# Autodesk Inventor assembly: richHolder
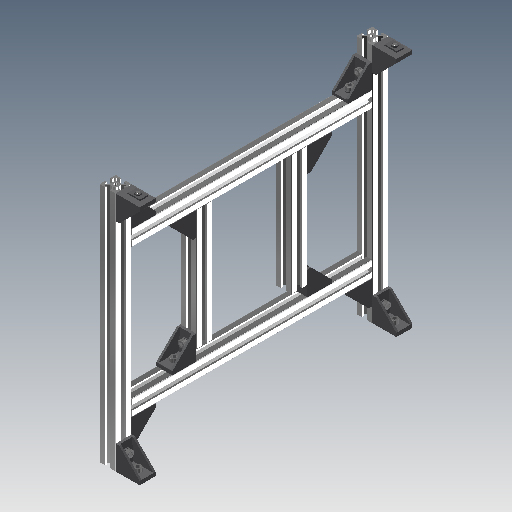
[picture p0: Inventor's stored thumbnail of the model, 512x512]
Saved by Autodesk Inventor 2018.2 (Build 222227000, 227)
## iProperties
Created: 2016-02-08
Part Number: richHolder
Document SubType Name: Assembly
Designer: Sawaiz
Author: Sawaiz
## Documents named in this file (6)
- C:\Users\sawaiz\OneDrive\projects\modularRICHFrame\frame\richHolder.iam
- C:\Users\sawaiz\OneDrive\projects\modularRICHFrame\hardware\angleBracket.iam
- C:\Users\sawaiz\OneDrive\projects\modularRICHFrame\frame\hfs5-2020Height.ipt
- C:\Users\sawaiz\OneDrive\projects\modularRICHFrame\frame\hfs5-2020Width.ipt
- C:\Users\sawaiz\OneDrive\projects\modularRICHFrame\frame\hfs5-2020BoxSeperator.ipt
- C:\Users\sawaiz\OneDrive\projects\modularRICHFrame\modularRICHFrame.xlsx
## Components (18 placed, 4 different names)
1. angleBracket:1 [sub-assembly] — Flush:30, Flush:31, Flush:35, Mate:19
2. angleBracket:2 [sub-assembly] — Flush:42, Flush:43, Mate:20
3. angleBracket:3 [sub-assembly] — Symmetry:4, Flush:33, Flush:34, Mate:21
4. angleBracket:4 [sub-assembly] — Symmetry:4, Flush:41, Flush:44, Mate:22
5. angleBracket:5 [sub-assembly] — Flush:6, Flush:7, Flush:10, Flush:12, Flush:32, Flush:50, Mate:24
6. angleBracket:6 [sub-assembly] — Flush:6, Flush:10, Flush:13, Flush:45, Flush:51, Mate:23
7. angleBracket:7 [sub-assembly] — Flush:5, Flush:7, Flush:9, Flush:12, Flush:36, Flush:48
8. angleBracket:8 [sub-assembly] — Flush:5, Flush:9, Flush:13, Flush:46, Flush:49, Mate:25
9. hfs5-2020Height:1 — Flush:30, Flush:31, Flush:42, Flush:43, Mate:19, Mate:20, Flush:47, Symmetry:5, Mate:26, Flush:52, Symmetry:8
10. hfs5-2020Height:2 — Flush:33, Flush:34, Flush:35, Flush:41, Flush:44, Mate:21, Mate:22, Flush:47, Symmetry:5, Mate:27, Symmetry:8
11. hfs5-2020Width:1 — Flush:45, Flush:46, Flush:49, Flush:51, Symmetry:6, Mate:23, Mate:25, Mate:31
12. hfs5-2020Width:2 — Flush:32, Flush:36, Flush:48, Flush:50, Symmetry:6, Mate:24, Mate:26, Mate:27, Flush:52, Flush:63, Mate:30
13. angleBracket:9 [sub-assembly] — Flush:22, Flush:26, Flush:39, Flush:54, Flush:55, Flush:61, Mate:29
14. angleBracket:10 [sub-assembly] — Flush:22, Flush:26, Flush:37, Flush:53, Flush:56, Flush:62, Mate:28
15. angleBracket:11 [sub-assembly] — Flush:24, Flush:27, Flush:40, Flush:54, Flush:60, Mate:31
16. angleBracket:12 [sub-assembly] — Flush:24, Flush:27, Flush:38, Flush:53, Flush:59
17. hfs5-2020BoxSeperator:1 — Flush:39, Flush:40, Symmetry:7, Flush:55, Flush:60, Flush:61, Mate:29
18. hfs5-2020BoxSeperator:2 — Flush:37, Flush:38, Symmetry:7, Flush:56, Flush:59, Flush:62, Mate:28, Flush:63, Mate:30
## Relationships (61: Flush 43, Mate 13, Symmetry 5)
- Flush:5: angleBracket:7 ↔ angleBracket:8
- Flush:6: angleBracket:5 ↔ angleBracket:6
- Flush:7: angleBracket:5 ↔ angleBracket:7
- Flush:9: angleBracket:7 ↔ angleBracket:8
- Flush:10: angleBracket:5 ↔ angleBracket:6
- Flush:12: angleBracket:5 ↔ angleBracket:7
- Flush:13: angleBracket:6 ↔ angleBracket:8
- Flush:22: angleBracket:9 ↔ angleBracket:10
- Flush:24: angleBracket:11 ↔ angleBracket:12
- Flush:26: angleBracket:9 ↔ angleBracket:10
- Flush:27: angleBracket:11 ↔ angleBracket:12
- Symmetry:4: angleBracket:3 ↔ angleBracket:4
- Flush:30: angleBracket:1 ↔ hfs5-2020Height:1
- Flush:31: angleBracket:1 ↔ hfs5-2020Height:1
- Flush:32: angleBracket:5 ↔ hfs5-2020Width:2
- Flush:33: angleBracket:3 ↔ hfs5-2020Height:2
- Flush:34: angleBracket:3 ↔ hfs5-2020Height:2
- Flush:35: angleBracket:1 ↔ hfs5-2020Height:2
- Flush:36: angleBracket:7 ↔ hfs5-2020Width:2
- Flush:37: angleBracket:10 ↔ hfs5-2020BoxSeperator:2
- Flush:38: angleBracket:12 ↔ hfs5-2020BoxSeperator:2
- Flush:39: angleBracket:9 ↔ hfs5-2020BoxSeperator:1
- Flush:40: angleBracket:11 ↔ hfs5-2020BoxSeperator:1
- Flush:41: angleBracket:4 ↔ hfs5-2020Height:2
- Flush:42: angleBracket:2 ↔ hfs5-2020Height:1
- Flush:43: angleBracket:2 ↔ hfs5-2020Height:1
- Flush:44: angleBracket:4 ↔ hfs5-2020Height:2
- Flush:45: angleBracket:6 ↔ hfs5-2020Width:1
- Flush:46: angleBracket:8 ↔ hfs5-2020Width:1
- Mate:19: angleBracket:1 ↔ hfs5-2020Height:1
- Mate:20: angleBracket:2 ↔ hfs5-2020Height:1
- Mate:21: angleBracket:3 ↔ hfs5-2020Height:2
- Mate:22: angleBracket:4 ↔ hfs5-2020Height:2
- Flush:47: hfs5-2020Height:1 ↔ hfs5-2020Height:2
- Symmetry:5: hfs5-2020Height:1 ↔ hfs5-2020Height:2
- Flush:48: angleBracket:7 ↔ hfs5-2020Width:2
- Flush:49: angleBracket:8 ↔ hfs5-2020Width:1
- Flush:50: angleBracket:5 ↔ hfs5-2020Width:2
- Flush:51: angleBracket:6 ↔ hfs5-2020Width:1
- Symmetry:6: hfs5-2020Width:1 ↔ hfs5-2020Width:2
- Symmetry:7: hfs5-2020BoxSeperator:1 ↔ hfs5-2020BoxSeperator:2
- Mate:23: angleBracket:6 ↔ hfs5-2020Width:1
- Mate:24: angleBracket:5 ↔ hfs5-2020Width:2
- Mate:25: angleBracket:8 ↔ hfs5-2020Width:1
- Mate:26: hfs5-2020Height:1 ↔ hfs5-2020Width:2
- Mate:27: hfs5-2020Height:2 ↔ hfs5-2020Width:2
- Flush:52: hfs5-2020Height:1 ↔ hfs5-2020Width:2
- Symmetry:8: hfs5-2020Height:1 ↔ hfs5-2020Height:2
- Flush:53: angleBracket:10 ↔ angleBracket:12
- Flush:54: angleBracket:9 ↔ angleBracket:11
- Flush:55: angleBracket:9 ↔ hfs5-2020BoxSeperator:1
- Flush:56: angleBracket:10 ↔ hfs5-2020BoxSeperator:2
- Flush:59: angleBracket:12 ↔ hfs5-2020BoxSeperator:2
- Flush:60: angleBracket:11 ↔ hfs5-2020BoxSeperator:1
- Flush:61: angleBracket:9 ↔ hfs5-2020BoxSeperator:1
- Flush:62: angleBracket:10 ↔ hfs5-2020BoxSeperator:2
- Mate:28: angleBracket:10 ↔ hfs5-2020BoxSeperator:2
- Mate:29: angleBracket:9 ↔ hfs5-2020BoxSeperator:1
- Flush:63: hfs5-2020Width:2 ↔ hfs5-2020BoxSeperator:2
- Mate:30: hfs5-2020Width:2 ↔ hfs5-2020BoxSeperator:2
- Mate:31: hfs5-2020Width:1 ↔ angleBracket:11
## Named parameters: frameAcrylicThickness = 9.525 mm, internalAcrylicThickness = 6.35 mm, aerogelThickness = 30 mm, aerogelWidth = 110 mm, aerogelHeight = 110 mm, height = 300 mm, width = 300 mm, depth = 500 mm, mirrorAngle = 5 deg, detectorWidth = 52 mm, detectorHeight = 52 mm, mirrorThickness = 3.175 mm, fresnelThickness = 0.1 mm, grooveDensity = 100, focalLength = 76.2 mm, ior = 1.49, centerThickness = 1.524 mm, fresnelAngle = 90 deg, fresnelEffectiveDiameter = 152.4 mm, oRingWidth = 1.5875 mm, sensorHolderDepth = 19.05 mm, aerogelClearence = 3.175 mm, backplanePCBWidth = 76.2 mm, backplanePCBHeight = 76.2 mm, backplaneHoleOffsett = 6.35 mm, backplanePostionOffsett = 12.7 mm, moduleSlotClearence = 0.79375 mm, testMountLength = 500 mm, testMountWidth = 300 mm, testMountHeight = 300 mm, facingThickness = 12.7 mm, facingGasketThickness = 1.5875 mm
